# Autodesk Inventor assembly: disk
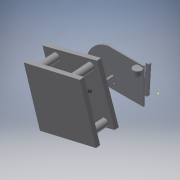
[picture p0: Inventor's stored thumbnail of the model, 180x180]
Saved by Autodesk Inventor 2019 (Build 230136000, 136)
## iProperties
Created: 2020-02-20
Part Number: disk
Document SubType Name: Assembly
Designer: ADMIN
Author: ADMIN
## Documents named in this file (10)
- E:\disk.iam
- F:\expo\holder.ipt
- F:\expo\glassplane.ipt
- F:\expo\rod.ipt
- F:\expo\wheel.ipt
- F:\expo\base1.ipt
- F:\expo\lowerbase.ipt
- F:\expo\stepper.ipt
- F:\expo\strip.ipt
- F:\expo\angle.ipt
## Components (9 placed, 9 different names)
1. holder:1
2. glassplane:1
3. rod:1 — Mate:1, Mate:2
4. wheel:1 — Mate:1
5. base1:1 — Mate:2
6. lowerbase:1
7. stepper:1
8. strip:1
9. angle:1
## Relationships (2: Mate 2)
- Mate:1: rod:1 ↔ wheel:1
- Mate:2: rod:1 ↔ base1:1
